# Autodesk Inventor assembly: FInal Cover Assembly
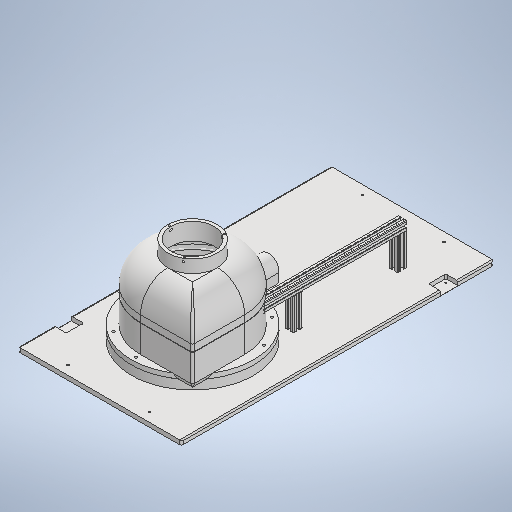
[picture p0: Inventor's stored thumbnail of the model, 512x512]
Saved by Autodesk Inventor 2025 (Build 290162000, 162)
## iProperties
Created: 2025-10-13
Part Number: FInal Cover Assembly
Document SubType Name: Assembly
Designer: mumin
Author: mumin
## Documents named in this file (10)
- C:\GitHub\In-situ-monitoring-of-powder-bed-fusion-additive-manufacturing\system_development\Orichalcum\v0.3\FInal Cover Assembly.iam
- C:\GitHub\In-situ-monitoring-of-powder-bed-fusion-additive-manufacturing\system_development\Orichalcum\v0.3\12mm Cover.ipt
- C:\GitHub\In-situ-monitoring-of-powder-bed-fusion-additive-manufacturing\system_development\Orichalcum\v0.3\SealedGlassRing.ipt
- C:\GitHub\In-situ-monitoring-of-powder-bed-fusion-additive-manufacturing\system_development\Orichalcum\v0.3\Cylinder Housing_base_3.ipt
- C:\GitHub\In-situ-monitoring-of-powder-bed-fusion-additive-manufacturing\system_development\Orichalcum\v0.3\Cylinder Housing_cap_3.ipt
- C:\GitHub\In-situ-monitoring-of-powder-bed-fusion-additive-manufacturing\system_development\Orichalcum\v0.3\2020 Legs (70mm).ipt
- C:\GitHub\In-situ-monitoring-of-powder-bed-fusion-additive-manufacturing\system_development\Orichalcum\v0.3\2020 LV-GVS Beam (481).ipt
- C:\GitHub\In-situ-monitoring-of-powder-bed-fusion-additive-manufacturing\system_development\Orichalcum\v0.3\GVS_Plate.ipt
- C:\GitHub\In-situ-monitoring-of-powder-bed-fusion-additive-manufacturing\system_development\Orichalcum\v0.3\GVS102-Step.ipt
- C:\GitHub\In-situ-monitoring-of-powder-bed-fusion-additive-manufacturing\system_development\Orichalcum\v0.3\CenterCylinder_2.ipt
## Components (10 placed, 9 different names)
1. 12mm Cover:1 — Insert:1, Insert:2, Insert:5, Insert:8
2. SealedGlassRing:1 — Insert:1, Insert:2, Insert:3, Insert:4
3. Cylinder Housing_base_3:1 — Insert:3, Insert:4, Mate:1, Flush:1, Flush:2
4. Cylinder Housing_cap_3:1 — Mate:1, Flush:1, Flush:2, Mate:4
5. 2020 Legs (70mm):1 — Insert:5, Flush:3, Mate:2, Flush:4
6. 2020 LV-GVS Beam (481):1 — Flush:3, Mate:2, Flush:4, Flush:5, Mate:3
7. GVS_Plate:1 — Flush:5, Mate:3, Insert:6, Insert:7
8. GVS102-Step:1 — Insert:6, Insert:7
9. CenterCylinder_2:1 — Mate:4
10. 2020 Legs (70mm):2 — Insert:8
## Relationships (17: Insert 8, Flush 5, Mate 4)
- Insert:1: 12mm Cover:1 ↔ SealedGlassRing:1
- Insert:2: 12mm Cover:1 ↔ SealedGlassRing:1
- Insert:3: SealedGlassRing:1 ↔ Cylinder Housing_base_3:1
- Insert:4: SealedGlassRing:1 ↔ Cylinder Housing_base_3:1
- Mate:1: Cylinder Housing_base_3:1 ↔ Cylinder Housing_cap_3:1
- Flush:1: Cylinder Housing_base_3:1 ↔ Cylinder Housing_cap_3:1
- Flush:2: Cylinder Housing_base_3:1 ↔ Cylinder Housing_cap_3:1
- Insert:5: 12mm Cover:1 ↔ 2020 Legs (70mm):1
- Flush:3: 2020 Legs (70mm):1 ↔ 2020 LV-GVS Beam (481):1
- Mate:2: 2020 Legs (70mm):1 ↔ 2020 LV-GVS Beam (481):1
- Flush:4: 2020 Legs (70mm):1 ↔ 2020 LV-GVS Beam (481):1
- Flush:5: 2020 LV-GVS Beam (481):1 ↔ GVS_Plate:1
- Mate:3: 2020 LV-GVS Beam (481):1 ↔ GVS_Plate:1
- Insert:6: GVS_Plate:1 ↔ GVS102-Step:1
- Insert:7: GVS_Plate:1 ↔ GVS102-Step:1
- Mate:4: Cylinder Housing_cap_3:1 ↔ CenterCylinder_2:1
- Insert:8: 12mm Cover:1 ↔ 2020 Legs (70mm):2
